# Autodesk Inventor assembly: BoronProbe
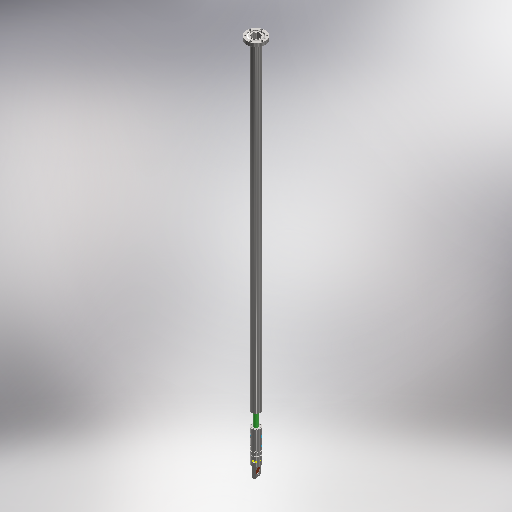
[picture p0: Inventor's stored thumbnail of the model, 512x512]
Saved by Autodesk Inventor 2026 (Build 300175050, 175E)
## iProperties
Created: 2025-07-13
Part Number: BoronProbe
Document SubType Name: Assembly
Designer: jin20
Author: jin20
## Documents named in this file (4)
- C:\Users\jin20\Documents\装置CAD\SpectroscopySystem\Probe\BoronProbe.iam
- C:\Users\jin20\Documents\装置CAD\PIHTI\BoronProbe\BoronProbe.iam
- C:\Users\jin20\Documents\装置CAD\PIHTI\BoronProbe\ProbeHead_hayashi\newversion\probe-head.iam
- C:\Users\jin20\OneDrive\ドキュメント\Inventor\Content Center Files\R2026\ja-JP\ISO 4762(2)\ISO 4762 - M4 x 12ISO.ipt
## Components (5 placed, 3 different names)
1. BoronProbe:1 [sub-assembly] — 挿入:1, 挿入:2, 挿入:3, 挿入:4, 挿入:5, 挿入:6
2. probe-head:1 [sub-assembly] — 挿入:4, 挿入:5, 挿入:6
3. ISO 4762 M4 x 12:3 — 挿入:2
4. ISO 4762 M4 x 12:1 — 挿入:1
5. ISO 4762 M4 x 12:2 — 挿入:3
## Relationships (6: Insert 6)
- 挿入:1 [Insert]: BoronProbe:1 ↔ ISO 4762 M4 x 12:1
- 挿入:2 [Insert]: BoronProbe:1 ↔ ISO 4762 M4 x 12:3
- 挿入:3 [Insert]: BoronProbe:1 ↔ ISO 4762 M4 x 12:2
- 挿入:4 [Insert]: BoronProbe:1 ↔ probe-head:1
- 挿入:5 [Insert]: BoronProbe:1 ↔ probe-head:1
- 挿入:6 [Insert]: BoronProbe:1 ↔ probe-head:1
